# Autodesk Inventor assembly: FRONT FRAME ASSEMBLY
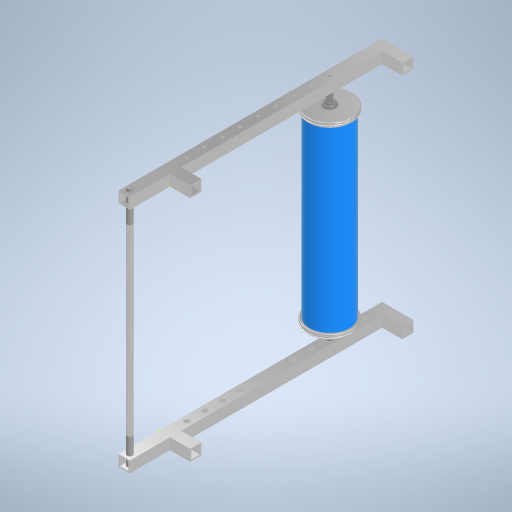
[picture p0: Inventor's stored thumbnail of the model, 512x512]
Saved by Autodesk Inventor 2023 (Build 270158000, 158)
## iProperties
Created: 2022-08-29
Part Number: FRONT FRAME ASSEMBLY
Document SubType Name: Assembly
Designer: D.C. Eksteen
Author: D.C. Eksteen
## Documents named in this file (5)
- C:\Users\dylan\Desktop\Skripsie-2022\Design\CAD\FRONT FRAME ASSEMBLY.iam
- C:\Users\dylan\Desktop\Skripsie-2022\Design\CAD\FRONT FRAME LEFT.iam
- C:\Users\dylan\Desktop\Skripsie-2022\Design\CAD\FRONT FRAME HINGE ROD.ipt
- C:\Users\dylan\Desktop\Skripsie-2022\Design\CAD\FRONT FRAME RIGHT.iam
- C:\Users\dylan\Desktop\Skripsie-2022\Design\CAD\IDLE ROLLER.iam
## Components (4 placed, 4 different names)
1. FRONT FRAME LEFT:1 [sub-assembly] — Mate:10, Mate:11
2. FRONT FRAME HINGE ROD:1
3. FRONT FRAME RIGHT:1 [sub-assembly] — Mate:8, Mate:9
4. IDLE ROLLER:1 [sub-assembly] — Mate:8, Mate:9
## Relationships (8: Mate 7, Flush 1)
- [Mate]: FRONT FRAME LEFT:1 ↔ FRONT FRAME HINGE ROD:1
- [Mate]: FRONT FRAME HINGE ROD:1 ↔ FRONT FRAME RIGHT:1
- [Flush]: FRONT FRAME LEFT:1 ↔ FRONT FRAME RIGHT:1
- [Mate] (530 mm): FRONT FRAME LEFT:1 ↔ FRONT FRAME RIGHT:1
- Mate:8: FRONT FRAME RIGHT:1 ↔ IDLE ROLLER:1
- Mate:9: FRONT FRAME RIGHT:1 ↔ IDLE ROLLER:1
- Mate:10: FRONT FRAME LEFT:1
- Mate:11: FRONT FRAME LEFT:1
